# Autodesk Inventor assembly: Крышка
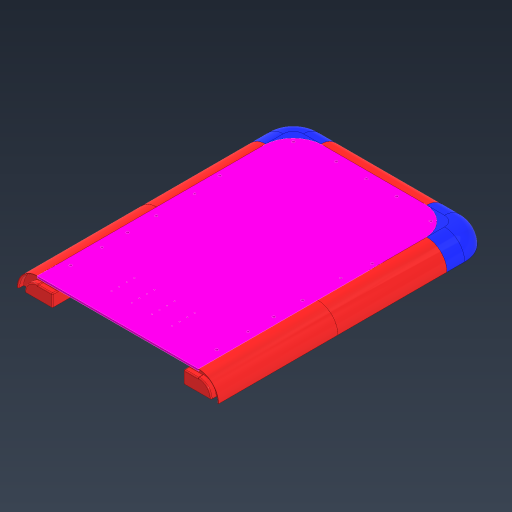
[picture p0: Inventor's stored thumbnail of the model, 512x512]
Saved by Autodesk Inventor 2023.2 (Build 272271030, 271C)
## iProperties
Created: 2025-05-05
Part Number: Крышка
Document SubType Name: Assembly
Designer: Олег Коноваленко
Author: Олег Коноваленко
## Documents named in this file (8)
- D:\!Rover\Rover\Rover_construction\Крышка.iam
- D:\!Rover\Rover\Rover_construction\Край задней части корпуса.ipt
- D:\!Rover\Rover\Rover_construction\кубик.ipt
- D:\!Rover\Rover\Rover_construction\Фанера_крышки.ipt
- D:\!Rover\Rover\Rover_construction\222LX-Konstruktsionnyy-profil-20kh20L.ipt
- D:\!Rover\Rover\Rover_construction\Край задней части корпуса_MIR.ipt
- D:\!Rover\Rover\Rover_construction\Край_новой_крышки.ipt
- D:\!Rover\Rover\Rover_construction\проставка.ipt
## Components (9 placed, 7 different names)
1. Край задней части корпуса:3 — Совмещение:3, Заподлицо:2, Совмещение:4, Совмещение:7, Совмещение:15, Совмещение:16, Совмещение:17, Совмещение:18, Совмещение:20, Совмещение:22, Совмещение:23, Совмещение:24, Заподлицо:8
2. кубик:1 — Совмещение:3, Заподлицо:2, Совмещение:4, Совмещение:19, Заподлицо:7
3. кубик:2 — Совмещение:14, Заподлицо:5
4. Фанера_крышки:1 — Совмещение:7, Совмещение:20, Совмещение:21
5. 222LX-Konstruktsionnyy-profil-20kh20L:1 — Совмещение:15, Совмещение:16, Совмещение:23
6. 222LX-Konstruktsionnyy-profil-20kh20L:2 — Совмещение:17, Совмещение:18, Совмещение:22
7. Край задней части корпуса_MIR:1 — Совмещение:14, Заподлицо:5
8. Край_новой_крышки:1 — Совмещение:19, Заподлицо:7, Совмещение:21
9. проставка:1 — Совмещение:24, Заподлицо:8
## Relationships (18: Mate 14, Flush 4)
- Совмещение:3 [Mate]: Край задней части корпуса:3 ↔ кубик:1
- Заподлицо:2 [Flush]: Край задней части корпуса:3 ↔ кубик:1
- Совмещение:4 [Mate]: Край задней части корпуса:3 ↔ кубик:1
- Совмещение:7 [Mate]: Край задней части корпуса:3 ↔ Фанера_крышки:1
- Совмещение:14 [Mate]: кубик:2 ↔ Край задней части корпуса_MIR:1
- Заподлицо:5 [Flush]: кубик:2 ↔ Край задней части корпуса_MIR:1
- Совмещение:15 [Mate] (1 mm): Край задней части корпуса:3 ↔ 222LX-Konstruktsionnyy-profil-20kh20L:1
- Совмещение:16 [Mate] (1 mm): Край задней части корпуса:3 ↔ 222LX-Konstruktsionnyy-profil-20kh20L:1
- Совмещение:17 [Mate] (1 mm): Край задней части корпуса:3 ↔ 222LX-Konstruktsionnyy-profil-20kh20L:2
- Совмещение:18 [Mate] (1 mm): Край задней части корпуса:3 ↔ 222LX-Konstruktsionnyy-profil-20kh20L:2
- Совмещение:19 [Mate]: кубик:1 ↔ Край_новой_крышки:1
- Заподлицо:7 [Flush]: кубик:1 ↔ Край_новой_крышки:1
- Совмещение:20 [Mate]: Край задней части корпуса:3 ↔ Фанера_крышки:1
- Совмещение:21 [Mate]: Фанера_крышки:1 ↔ Край_новой_крышки:1
- Совмещение:22 [Mate]: Край задней части корпуса:3 ↔ 222LX-Konstruktsionnyy-profil-20kh20L:2
- Совмещение:23 [Mate]: Край задней части корпуса:3 ↔ 222LX-Konstruktsionnyy-profil-20kh20L:1
- Совмещение:24 [Mate]: Край задней части корпуса:3 ↔ проставка:1
- Заподлицо:8 [Flush]: Край задней части корпуса:3 ↔ проставка:1
